# Autodesk Inventor assembly: WasherAssembly
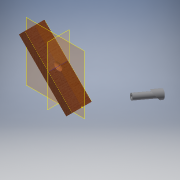
[picture p0: Inventor's stored thumbnail of the model, 180x180]
Saved by Autodesk Inventor 2019.4 (Build 234330000, 330)
## iProperties
Created: 2019-06-16
Part Number: WasherAssembly
Document SubType Name: Assembly
Designer: steele
Author: steele
## Documents named in this file (3)
- C:\git\CAD-Development\robSteele\HouseProjects\ElectricFenceWasher\WasherAssembly.iam
- C:\git\CAD-Development\robSteele\HouseProjects\ElectricFenceWasher\2x4x12.ipt
- C:\git\CAD-Development\robSteele\HouseProjects\ElectricFenceWasher\Whack03.ipt
## Components (2 placed, 2 different names)
1. 2x4x12:1 — Flush:2
2. Whack03:1 — Flush:2
## Relationships (1: Flush 1)
- Flush:2: 2x4x12:1 ↔ Whack03:1
